# Autodesk Inventor assembly: switch assembly
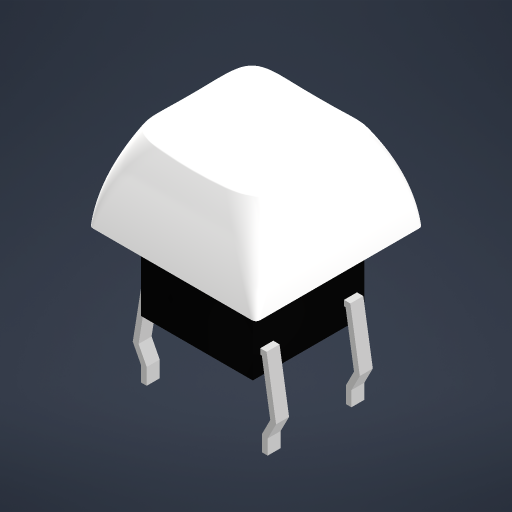
[picture p0: Inventor's stored thumbnail of the model, 512x512]
Saved by Autodesk Inventor 2024.2 (Build 282272000, 272)
## iProperties
Created: 2024-12-04
Part Number: switch assembly
Document SubType Name: Assembly
Designer: Moe
Author: Moe
## Documents named in this file (3)
- D:\Code\git\tiny-keeb\caps\switch assembly.iam
- D:\Code\git\tiny-keeb\caps\switch ref\b3f-1050.iam
- D:\Code\git\tiny-keeb\caps\cap ref\1u.ipt
## Components (2 placed, 2 different names)
1. b3f-1050:1 [sub-assembly] — Mate:1
2. 1u:1 — Mate:1
## Relationships (1: Mate 1)
- Mate:1: b3f-1050:1 ↔ 1u:1
